# Autodesk Inventor assembly: TreadAssembly
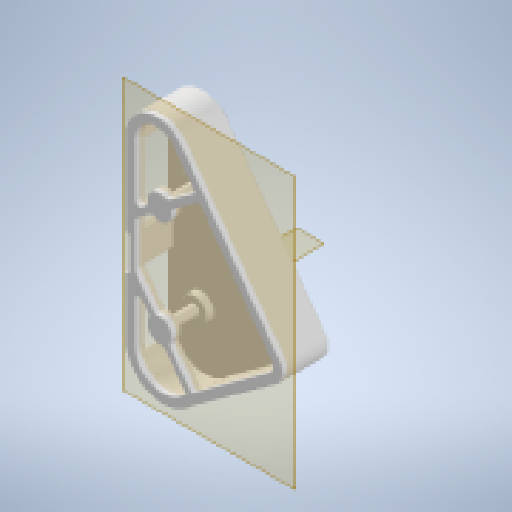
[picture p0: Inventor's stored thumbnail of the model, 512x512]
Saved by Autodesk Inventor 2025.2 (Build 292293000, 293)
## iProperties
Created: 2025-01-27
Part Number: TreadAssembly
Document SubType Name: Assembly
Designer: andre
Author: andre
## Documents named in this file (3)
- C:\Users\andre\Documents\GitHub\Handshake\Hardware\Proto2-WallE\TreadAssembly.iam
- C:\Users\andre\Documents\GitHub\Handshake\Hardware\Proto2-WallE\TreadWheeled.ipt
- C:\Users\andre\Documents\GitHub\Handshake\Hardware\Proto2-WallE\TreadWheeledCover.ipt
## Components (2 placed, 2 different names)
1. TreadWheeled:1 — Flush:1, Flush:2
2. TreadWheeledCover:1 — Flush:1, Flush:2
## Relationships (2: Flush 2)
- Flush:1: TreadWheeled:1 ↔ TreadWheeledCover:1
- Flush:2: TreadWheeled:1 ↔ TreadWheeledCover:1
